# Autodesk Inventor assembly: mcu_board
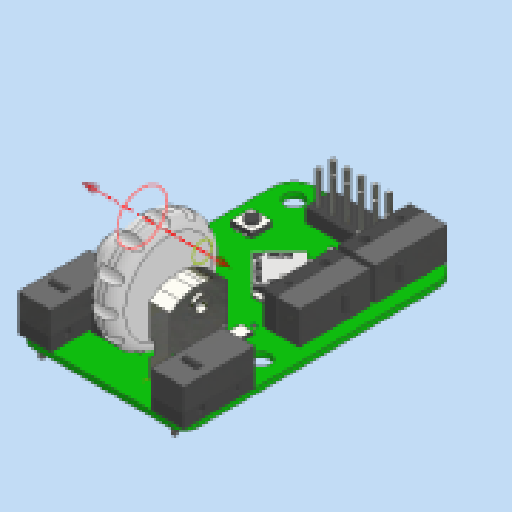
[picture p0: Inventor's stored thumbnail of the model, 512x512]
Saved by Autodesk Inventor 2024 (Build 280153000, 153)
## iProperties
Created: 2025-05-06
Part Number: mcu_board
Document SubType Name: Assembly
Designer: XxPan
Author: XxPan
## iProperties of the stored document 44PW_ATM.ipt
Created: 2025-05-06
Part Number: product
Material: Generic
Description: STEP AP214
Document SubType Name: Modeling
Designer: XxPan
Density: 1 g/cm^3
Appearance: Default
Title: 44PW_ATM
Revision Number: 1.0first version
## iProperties of the stored document CAP_0201.ipt
Created: 2024-08-04
Part Number: GRM_Auto_Q3_0.6_0.3_0.33_0.15
Material: Generic
Description: STEP AP214
Document SubType Name: Modeling
Designer: XxPan
Density: 1 g/cm^3
Appearance: Default
Sending System: SolidWorks 2021
Preprocessor: SwSTEP 2.0
Title: GRM_Auto_Q3_0.6_0.3_0.33_0.15.STEP
Revision Number: ANY
## Documents named in this file (18)
- D:\The Mind Palace\remmy_mouse\CAD\mcu_board.iam
- **D:\The Mind Palace\remmy_mouse\CAD\mcu_board.iam*LocalDocs*xAaaaaddaAaaaaaaaAaaaajjlXb*44PW_ATM.ipt
- D:\The Mind Palace\remmy_mouse\CAD\6mm_switch.ipt
- D:\The Mind Palace\remmy_mouse\CAD\Kailh_GM_8.0_switch.ipt
- D:\The Mind Palace\remmy_mouse\CAD\TTC_silver_rotary_encoder.ipt
- D:\The Mind Palace\remmy_mouse\CAD\mcu_pcb.ipt
- D:\The Mind Palace\remmy_mouse\CAD\crystal_oscillator.ipt
- **D:\The Mind Palace\remmy_mouse\CAD\mcu_board.iam*LocalDocs*xAaaaqxcaAaaaaaaaAaaaamazQe*CAP_0201.ipt
- D:\The Mind Palace\remmy_mouse\CAD\scroll_wheel.ipt
- D:\The Mind Palace\remmy_mouse\CAD\2x5_P2.54mm_male_header.ipt
- D:\The Mind Palace\remmy_mouse\CAD\mcu_label.ipt
- D:\The Mind Palace\remmy_mouse\CAD\R-667842_tactile_switch.ipt
- D:\The Mind Palace\remmy_mouse\CAD\scroll_wheel_axle.ipt
- D:\The Mind Palace\remmy_mouse\CAD\shell\scroll_wheel_with_axle.ipt
- **C:\Users\XxPan\OneDrive - McMaster University\Mouse\CAD\mcu_board.iam*LocalDocs*xAaaaaddaAaaaaaaaAaaaajjlXb*44PW_ATM.ipt
- **C:\Users\XxPan\OneDrive - McMaster University\Mouse\CAD\mcu_board.iam*LocalDocs*xAaaaqxcaAaaaaaaaAaaaamazQe*CAP_0201.ipt
- D:\The Mind Palace\remmy_mouse\CAD_models\ATMEGA32U4_MU\44PW_ATM.step
- D:\The Mind Palace\remmy_mouse\CAD_models\capacitors\CAP_0201.step
## Components (18 placed, 13 different names)
1. 44PW_ATM:1 — Mate:1, Flush:6, Mate:23, Flush:7, Angle:1
2. 6mm_switch:1 — Mate:5, Mate:30, Flush:24
3. TTC_silver_rotary_encoder:1 — Mate:4, Insert:3, Flush:22, Flush:23, Insert:4
4. mcu_pcb:1 — Mate:1, Mate:2, Mate:3, Mate:4, Mate:5, Mate:6, Mate:9, Mate:10, Mate:20, Mate:22, Angle:1, Mate:25, Mate:26, Flush:12, Flush:13, Mate:27, Flush:16, Flush:18, Flush:19, Flush:20, Flush:21, Flush:22, Flush:23, Flush:24, Flush:25, Flush:26, Flush:27, Flush:28, Flush:29, Flush:30
5. Kailh_GM_8.0_switch:2 — Mate:21, Flush:4, Flush:5, Mate:27
6. Kailh_GM_8.0_switch:3 — Mate:21, Flush:4, Flush:5, Mate:22, Flush:16
7. Kailh_GM_8.0_switch:1 — Mate:2, Flush:18, Flush:19
8. Kailh_GM_8.0_switch:4 — Mate:3, Flush:20, Flush:21
9. crystal_oscillator:1 — Mate:6, Mate:13, Mate:14, Flush:1, Flush:2
10. CAP_0201:1 — Mate:10, Mate:13, Flush:2
11. CAP_0201:2 — Mate:9, Mate:14, Flush:1
12. scroll_wheel:1 — Angle:2, Flush:17, Mate:28, Angle:3, Insert:3, Mate:30
13. 2x5_P2.54mm_male_header:1 — Mate:20, Flush:30
14. mcu_label:1 — Flush:6, Mate:23, Flush:7
15. R-667842_tactile_switch:2 — Mate:26, Flush:25, Flush:26
16. R-667842_tactile_switch:1 — Mate:25, Flush:12, Flush:13
17. scroll_wheel_axle:1 — Flush:17, Mate:28, Angle:3
18. scroll_wheel_with_axle:1 — Insert:4
## Relationships (47: Flush 23, Mate 19, Angle 3, Insert 2)
- Mate:1: 44PW_ATM:1 ↔ mcu_pcb:1
- Mate:2: mcu_pcb:1 ↔ Kailh_GM_8.0_switch:1
- Mate:3: mcu_pcb:1 ↔ Kailh_GM_8.0_switch:4
- Mate:4: TTC_silver_rotary_encoder:1 ↔ mcu_pcb:1
- Mate:5: 6mm_switch:1 ↔ mcu_pcb:1
- Mate:6: mcu_pcb:1 ↔ crystal_oscillator:1
- Mate:9: mcu_pcb:1 ↔ CAP_0201:2
- Mate:10: mcu_pcb:1 ↔ CAP_0201:1
- Mate:13 (1 mm): crystal_oscillator:1 ↔ CAP_0201:1
- Mate:14 (1 mm): crystal_oscillator:1 ↔ CAP_0201:2
- Flush:1 (-1 mm): crystal_oscillator:1 ↔ CAP_0201:2
- Flush:2 (1 mm): crystal_oscillator:1 ↔ CAP_0201:1
- Mate:20: mcu_pcb:1 ↔ 2x5_P2.54mm_male_header:1
- Mate:21 (1 mm): Kailh_GM_8.0_switch:2 ↔ Kailh_GM_8.0_switch:3
- Flush:4: Kailh_GM_8.0_switch:2 ↔ Kailh_GM_8.0_switch:3
- Flush:5: Kailh_GM_8.0_switch:2 ↔ Kailh_GM_8.0_switch:3
- Mate:22 (8 mm): mcu_pcb:1 ↔ Kailh_GM_8.0_switch:3
- Flush:6: 44PW_ATM:1 ↔ mcu_label:1
- Mate:23: 44PW_ATM:1 ↔ mcu_label:1
- Flush:7: 44PW_ATM:1 ↔ mcu_label:1
- Angle:1 (45 deg): 44PW_ATM:1 ↔ mcu_pcb:1
- Angle:2 (0 deg): scroll_wheel:1
- Mate:25: mcu_pcb:1 ↔ R-667842_tactile_switch:1
- Mate:26: mcu_pcb:1 ↔ R-667842_tactile_switch:2
- Flush:12 (1.8 mm): mcu_pcb:1 ↔ R-667842_tactile_switch:1
- Flush:13 (16.9 mm): mcu_pcb:1 ↔ R-667842_tactile_switch:1
- Mate:27 (-1 mm): mcu_pcb:1 ↔ Kailh_GM_8.0_switch:2
- Flush:16 (8 mm): mcu_pcb:1 ↔ Kailh_GM_8.0_switch:3
- Flush:17 (-0.5 mm): scroll_wheel:1 ↔ scroll_wheel_axle:1
- Mate:28: scroll_wheel:1 ↔ scroll_wheel_axle:1
- Angle:3 (0 deg): scroll_wheel:1 ↔ scroll_wheel_axle:1
- Flush:18: mcu_pcb:1 ↔ Kailh_GM_8.0_switch:1
- Flush:19: mcu_pcb:1 ↔ Kailh_GM_8.0_switch:1
- Flush:20: mcu_pcb:1 ↔ Kailh_GM_8.0_switch:4
- Flush:21: mcu_pcb:1 ↔ Kailh_GM_8.0_switch:4
- Insert:3 (5 mm): TTC_silver_rotary_encoder:1 ↔ scroll_wheel:1
- Mate:30: 6mm_switch:1 ↔ scroll_wheel:1
- Flush:22 (10 mm): TTC_silver_rotary_encoder:1 ↔ mcu_pcb:1
- Flush:23 (9.6 mm): TTC_silver_rotary_encoder:1 ↔ mcu_pcb:1
- Flush:24 (9.3 mm): 6mm_switch:1 ↔ mcu_pcb:1
- Flush:25 (3.2 mm): mcu_pcb:1 ↔ R-667842_tactile_switch:2
- Flush:26 (10 mm): mcu_pcb:1 ↔ R-667842_tactile_switch:2
- Flush:27: mcu_pcb:1
- Flush:28: mcu_pcb:1
- Flush:29: mcu_pcb:1
- Flush:30 (2.4 mm): mcu_pcb:1 ↔ 2x5_P2.54mm_male_header:1
- Insert:4 (-16 mm): TTC_silver_rotary_encoder:1 ↔ scroll_wheel_with_axle:1
